# Autodesk Inventor assembly: Motor Assembly
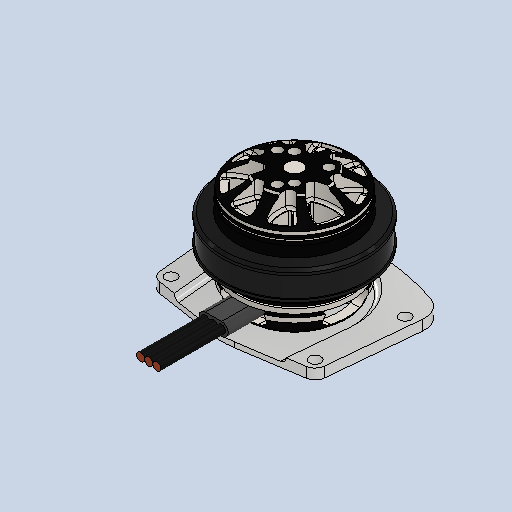
[picture p0: Inventor's stored thumbnail of the model, 512x512]
Saved by Autodesk Inventor 2023.2 (Build 272271000, 271)
## iProperties
Created: 2022-12-29
Part Number: Motor Assembly
Document SubType Name: Assembly
Designer: Nathan Cai
Mass: 123.954 g
Surface Area: 232.499 cm^2
Volume: 31.2781 cm^3
Density: 3.96298 g/cm^3
Author: Nathan Cai
## Documents named in this file (4)
- E:\Documents\Inventor\Moon Cake V1.01\Motor Assembly.iam
- E:\Documents\Inventor\Moon Cake V1.01\Motor Plate.ipt
- E:\Documents\Inventor\Moon Cake V1.01\Band - Hub.ipt
- E:\Documents\Inventor\Moon Cake V1.01\Flash_Hobby_D3536EVO v3\Flash_Hobby_D3536EVO v3.iam
## Components (3 placed, 3 different names)
1. Motor Plate:1 — Mate:26, Mate:27, Mate:28, Mate:29
2. Band - Hub:1 — Mate:26
3. Flash_Hobby_D3536EVO v3:1 [sub-assembly] — Mate:27, Mate:28, Mate:29
## Relationships (4: Mate 4)
- Mate:26 (12.7 mm): Motor Plate:1 ↔ Band - Hub:1
- Mate:27: Motor Plate:1 ↔ Flash_Hobby_D3536EVO v3:1
- Mate:28: Motor Plate:1 ↔ Flash_Hobby_D3536EVO v3:1
- Mate:29: Motor Plate:1 ↔ Flash_Hobby_D3536EVO v3:1
